# Autodesk Inventor assembly: EV-PE4312-EK
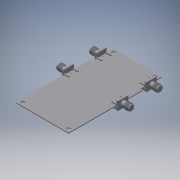
[picture p0: Inventor's stored thumbnail of the model, 180x180]
Saved by Autodesk Inventor 2018 (Build 220112000, 112)
## iProperties
Created: 2018-04-06
Part Number: EV-PE4312-EK
Document SubType Name: Assembly
Designer: bbramman
Author: bbramman
## Documents named in this file (3)
- C:\Users\bbramman\OneDrive\Documents\Trapped Ion Research (Grad)\Electronics\pll-evalboard-synthesizer\Box CAD\EV-PE4312-EK.iam
- C:\Users\bbramman\OneDrive\Documents\Trapped Ion Research (Grad)\Electronics\pll-evalboard-synthesizer\Box CAD\89x49mm-PCB.ipt
- C:\Users\bbramman\OneDrive\Documents\Trapped Ion Research (Grad)\Electronics\pll-evalboard-synthesizer\Box CAD\SMA-END.ipt
## Components (5 placed, 2 different names)
1. 89x49mm-PCB:1 — Mate:1, Mate:2, Mate:3, Mate:4, Mate:5, Mate:6, Mate:7, Mate:8, Flush:1, Flush:2, Flush:3, Flush:4
2. SMA-END:1 — Mate:2, Mate:8, Flush:1
3. SMA-END:2 — Mate:1, Mate:7, Flush:4
4. SMA-END:3 — Mate:4, Mate:6, Flush:2
5. SMA-END:4 — Mate:3, Mate:5, Flush:3
## Relationships (12: Mate 8, Flush 4)
- Mate:1: 89x49mm-PCB:1 ↔ SMA-END:2
- Mate:2: 89x49mm-PCB:1 ↔ SMA-END:1
- Mate:3: 89x49mm-PCB:1 ↔ SMA-END:4
- Mate:4: 89x49mm-PCB:1 ↔ SMA-END:3
- Mate:5: 89x49mm-PCB:1 ↔ SMA-END:4
- Mate:6: 89x49mm-PCB:1 ↔ SMA-END:3
- Mate:7: 89x49mm-PCB:1 ↔ SMA-END:2
- Mate:8: 89x49mm-PCB:1 ↔ SMA-END:1
- Flush:1 (6.35 mm): 89x49mm-PCB:1 ↔ SMA-END:1
- Flush:2 (6.35 mm): 89x49mm-PCB:1 ↔ SMA-END:3
- Flush:3 (34.925 mm): 89x49mm-PCB:1 ↔ SMA-END:4
- Flush:4 (34.925 mm): 89x49mm-PCB:1 ↔ SMA-END:2
